# Autodesk Inventor assembly: #Spindexer
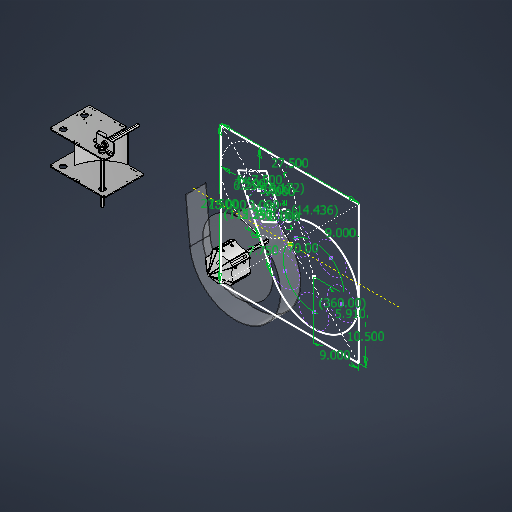
[picture p0: Inventor's stored thumbnail of the model, 512x512]
Saved by Autodesk Inventor 2026 (Build 300175000, 175)
## iProperties
Created: 2026-02-05
Part Number: #Spindexer
Document SubType Name: Assembly
Designer: Owen L
Author: Owen L
## Documents named in this file (15)
- C:\Users\littl\OneDrive\Documents\GitHub\2026-Robot-Mechanical\Spindexer\#Spindexer.iam
- C:\Users\littl\OneDrive\Documents\GitHub\2026-Robot-Mechanical\Spindexer\TEMP,BASE-SKETCH.ipt
- C:\Users\littl\OneDrive\Documents\GitHub\2026-Robot-Mechanical\Spindexer\3DPRINT,HUB.ipt
- C:\Users\littl\OneDrive\Documents\GitHub\2026-Robot-Mechanical\Spindexer\3DPRINT,HUB,CONE.ipt
- C:\Users\littl\OneDrive\Documents\GitHub\2026-Robot-Mechanical\Spindexer\PLATE,WALL.ipt
- C:\Users\littl\OneDrive\Documents\GitHub\2026-Robot-Mechanical\Spindexer\PLATE,BOTTOM.ipt
- C:\Users\littl\OneDrive\Documents\GitHub\2026-Robot-Mechanical\Spindexer\STOCK,HEX,SHAFT,HUB.ipt
- C:\Users\littl\OneDrive\Documents\GitHub\2026-Robot-Mechanical\Spindexer\STOCK,HEX,SHAFT,OUTPUT.ipt
- C:\Users\littl\OneDrive\Documents\GitHub\2026-Robot-Mechanical\Spindexer\TEMP,BASE-SKETCH,TANGENT-OUT.ipt
- C:\Users\littl\OneDrive\Documents\GitHub\2026-Robot-Mechanical\Spindexer\PLATE,KICKER,OUTSIDE.ipt
- C:\Users\littl\OneDrive\Documents\GitHub\2026-Robot-Mechanical\Spindexer\3DPRINT,KICKER,RAMP.ipt
- C:\Users\littl\OneDrive\Documents\GitHub\2026-Robot-Mechanical\Spindexer\PLATE,KICKER,INSIDE.ipt
- C:\Users\littl\OneDrive\Documents\GitHub\2026-Robot-Mechanical\Spindexer\PLATE,VERTICAL,ROLLER,BRACKET.ipt
- C:\Users\littl\OneDrive\Documents\GitHub\2026-Robot-Mechanical\Spindexer\PURCHASED,20T,HEX,MITER,GEAR.ipt
- C:\Users\littl\OneDrive\Documents\GitHub\2026-Robot-Mechanical\Spindexer\STOCK,HEX,SHAFT,VERTICAL.ipt
## Components (15 placed, 14 different names)
1. TEMP,BASE-SKETCH:1
2. 3DPRINT,HUB:1 — Mate:11, Mate:12, Mate:13, Mate:15, Mate:16, Mate:17, Flush:2, Mate:18, Mate:19, Mate:20
3. 3DPRINT,HUB,CONE:1 — Mate:11, Mate:12, Mate:13
4. PLATE,WALL:1
5. PLATE,BOTTOM:1 — Mate:18, Mate:19, Mate:20
6. STOCK,HEX,SHAFT,HUB:1 — Mate:16, Mate:17, Flush:2
7. STOCK,HEX,SHAFT,OUTPUT:1 — Mate:27, Mate:28
8. TEMP,BASE-SKETCH,TANGENT-OUT:1
9. PLATE,KICKER,OUTSIDE:1 — Mate:22, Mate:23, Mate:24, Mate:25, Flush:3, Flush:4
10. 3DPRINT,KICKER,RAMP:1 — Mate:22, Mate:23, Mate:24
11. PLATE,KICKER,INSIDE:1 — Mate:25, Flush:3, Flush:4, Mate:26, Flush:5, Flush:6, Mate:27
12. PLATE,VERTICAL,ROLLER,BRACKET:1 — Mate:26, Flush:5, Flush:6, Mate:29
13. PURCHASED,20T,HEX,MITER,GEAR:1 — Mate:28
14. PURCHASED,20T,HEX,MITER,GEAR:2 — Mate:30
15. STOCK,HEX,SHAFT,VERTICAL:1 — Mate:29, Mate:30
## Relationships (23: Mate 18, Flush 5)
- Mate:11: 3DPRINT,HUB:1 ↔ 3DPRINT,HUB,CONE:1
- Mate:12: 3DPRINT,HUB:1 ↔ 3DPRINT,HUB,CONE:1
- Mate:13: 3DPRINT,HUB:1 ↔ 3DPRINT,HUB,CONE:1
- Mate:15: 3DPRINT,HUB:1
- Mate:16: 3DPRINT,HUB:1 ↔ STOCK,HEX,SHAFT,HUB:1
- Mate:17: 3DPRINT,HUB:1 ↔ STOCK,HEX,SHAFT,HUB:1
- Flush:2 (-12.7 mm): 3DPRINT,HUB:1 ↔ STOCK,HEX,SHAFT,HUB:1
- Mate:18: 3DPRINT,HUB:1 ↔ PLATE,BOTTOM:1
- Mate:19: 3DPRINT,HUB:1 ↔ PLATE,BOTTOM:1
- Mate:20: 3DPRINT,HUB:1 ↔ PLATE,BOTTOM:1
- Mate:22: PLATE,KICKER,OUTSIDE:1 ↔ 3DPRINT,KICKER,RAMP:1
- Mate:23: PLATE,KICKER,OUTSIDE:1 ↔ 3DPRINT,KICKER,RAMP:1
- Mate:24: PLATE,KICKER,OUTSIDE:1 ↔ 3DPRINT,KICKER,RAMP:1
- Mate:25 (158.75 mm): PLATE,KICKER,OUTSIDE:1 ↔ PLATE,KICKER,INSIDE:1
- Flush:3: PLATE,KICKER,OUTSIDE:1 ↔ PLATE,KICKER,INSIDE:1
- Flush:4: PLATE,KICKER,OUTSIDE:1 ↔ PLATE,KICKER,INSIDE:1
- Mate:26: PLATE,KICKER,INSIDE:1 ↔ PLATE,VERTICAL,ROLLER,BRACKET:1
- Flush:5: PLATE,KICKER,INSIDE:1 ↔ PLATE,VERTICAL,ROLLER,BRACKET:1
- Flush:6: PLATE,KICKER,INSIDE:1 ↔ PLATE,VERTICAL,ROLLER,BRACKET:1
- Mate:27: STOCK,HEX,SHAFT,OUTPUT:1 ↔ PLATE,KICKER,INSIDE:1
- Mate:28: STOCK,HEX,SHAFT,OUTPUT:1 ↔ PURCHASED,20T,HEX,MITER,GEAR:1
- Mate:29: PLATE,VERTICAL,ROLLER,BRACKET:1 ↔ STOCK,HEX,SHAFT,VERTICAL:1
- Mate:30: PURCHASED,20T,HEX,MITER,GEAR:2 ↔ STOCK,HEX,SHAFT,VERTICAL:1
